# Autodesk Inventor assembly: caliber_truck
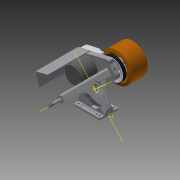
[picture p0: Inventor's stored thumbnail of the model, 180x180]
Saved by Autodesk Inventor 2014 (Build 180170000, 170)
## iProperties
Created: 2014-02-23
Part Number: caliber_truck
Document SubType Name: Assembly
Designer: Brent Yi
Author: Brent Yi
## Documents named in this file (10)
- C:\Users\brent\Documents\electric-longboard\brent\truck.iam
- C:\Users\brent\Documents\electric-longboard\brent\baseplate.ipt
- C:\Users\brent\Documents\electric-longboard\brent\hanger.ipt
- C:\Users\brent\Documents\electric-longboard\brent\mount_alt.ipt
- C:\Users\brent\Documents\electric-longboard\brent\wheel90mmwithbearing.iam
- C:\Users\brent\Documents\electric-longboard\brent\6354motor.ipt
- C:\Users\brent\Documents\electric-longboard\brent\Imported Components\15t_pulley\15t_pulley.ipt
- C:\Users\brent\Documents\electric-longboard\brent\motorguard.ipt
- C:\Users\brent\Documents\electric-longboard\brent\pulleyprotector.ipt
- C:\Users\brent\Documents\electric-longboard\brent\belt.ipt
## Components (10 placed, 9 different names)
1. baseplate:1 — Mate:1, Mate:2, Mate:17, Mate:30, Mate:31, Mate:35
2. hanger:1 — Mate:1, Mate:2, Mate:7, Mate:9, Mate:16, Flush:1, Mate:25, Mate:28, Mate:32, Mate:33, Mate:46
3. wheel90mmwithbearing:1 [sub-assembly] — Mate:7, Mate:25
4. wheel90mmwithbearing:2 [sub-assembly] — Mate:9, Mate:28
5. mount_alt:1 — Flush:1, Mate:21, Mate:32, Mate:33, Mate:34, Mate:41, Mate:42, Flush:3, Mate:49, Mate:50, Mate:51
6. 6354motor:1 — Mate:21, Mate:23, Mate:26, Mate:34, Mate:47
7. 15t_pulley:1 — Mate:23, Mate:26, Mate:48
8. motorguard:1 — Mate:41, Mate:42, Flush:3
9. pulleyprotector:1 — Mate:49, Mate:50, Mate:51
10. belt:1 — Mate:46, Mate:47, Mate:48
## Relationships (27: Mate 25, Flush 2)
- Mate:1: baseplate:1 ↔ hanger:1
- Mate:2: baseplate:1 ↔ hanger:1
- Mate:7: hanger:1 ↔ wheel90mmwithbearing:1
- Mate:9: hanger:1 ↔ wheel90mmwithbearing:2
- Mate:16: hanger:1
- Mate:17: baseplate:1
- Flush:1 (-28.575 mm): hanger:1 ↔ mount_alt:1
- Mate:21: mount_alt:1 ↔ 6354motor:1
- Mate:23: 6354motor:1 ↔ 15t_pulley:1
- Mate:25 (1.27 mm): hanger:1 ↔ wheel90mmwithbearing:1
- Mate:26 (5.08 mm): 6354motor:1 ↔ 15t_pulley:1
- Mate:28 (1.27 mm): hanger:1 ↔ wheel90mmwithbearing:2
- Mate:30: baseplate:1
- Mate:31: baseplate:1
- Mate:32: hanger:1 ↔ mount_alt:1
- Mate:33: hanger:1 ↔ mount_alt:1
- Mate:34: mount_alt:1 ↔ 6354motor:1
- Mate:35: baseplate:1
- Mate:41: mount_alt:1 ↔ motorguard:1
- Mate:42: mount_alt:1 ↔ motorguard:1
- Flush:3: mount_alt:1 ↔ motorguard:1
- Mate:46: hanger:1 ↔ belt:1
- Mate:47: 6354motor:1 ↔ belt:1
- Mate:48 (1 mm): 15t_pulley:1 ↔ belt:1
- Mate:49: mount_alt:1 ↔ pulleyprotector:1
- Mate:50: mount_alt:1 ↔ pulleyprotector:1
- Mate:51: mount_alt:1 ↔ pulleyprotector:1
